# Autodesk Inventor assembly: Pendolo_Inverso
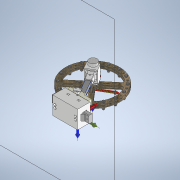
[picture p0: Inventor's stored thumbnail of the model, 180x180]
Saved by Autodesk Inventor 2020.2 (Build 242310000, 310)
## iProperties
Created: 2019-11-10
Part Number: Pendolo_Inverso
Document SubType Name: Assembly
Designer: socci
Author: socci
## Documents named in this file (27)
- C:\Users\socci\Desktop\mv-Project\04_PartDraw\Pendolo_Inverso.iam
- C:\Users\socci\Desktop\mv-Project\04_PartDraw\Componenti\19_Base_Pezzo_Unico.ipt
- C:\Users\socci\Documents\Inventor\Content Center Files\R2020\it-IT\Bearing GB_T 5800-2003\Rolling bearing GB_T 5800-2003 -635.ipt
- C:\Users\socci\Desktop\mv-Project\04_PartDraw\Componenti\1_Asse_cuscinetti.ipt
- C:\Users\socci\Desktop\mv-Project\04_PartDraw\Componenti\2_Connettore_inf_sup.ipt
- C:\Users\socci\Desktop\mv-Project\04_PartDraw\Componenti\3_Connettore_inf_INF.ipt
- C:\Users\socci\Desktop\mv-Project\04_PartDraw\Componenti\11_Connettore_MPU.ipt
- C:\Users\socci\Desktop\mv-Project\04_PartDraw\Componenti\10_MPU_6050.ipt
- C:\Users\socci\Desktop\mv-Project\04_PartDraw\Componenti\20_Base_Sopra.ipt
- C:\Users\socci\Desktop\mv-Project\04_PartDraw\Componenti\4_barra.ipt
- C:\Users\socci\Desktop\mv-Project\04_PartDraw\Componenti\22_Blocco_Escursione_Braccio.ipt
- C:\Users\socci\Desktop\mv-Project\04_PartDraw\Componenti\9_Flangia.ipt
- C:\Users\socci\Desktop\mv-Project\04_PartDraw\Componenti\24_Disco.ipt
- C:\Users\socci\Desktop\mv-Project\04_PartDraw\Componenti\26_Collana_di_Sfere.ipt
- C:\Users\socci\Documents\Inventor\Content Center Files\R2020\it-IT\DIN 1587\DIN 1587 - M6 x 1.ipt
- C:\Users\socci\Documents\Inventor\Content Center Files\R2020\it-IT\DIN 934\DIN 934 - M6 x 1.ipt
- C:\Users\socci\Desktop\mv-Project\04_PartDraw\Componenti\28_Rondella_M6.ipt
- C:\Users\socci\Documents\Inventor\Content Center Files\R2020\it-IT\DIN 933\DIN 933 - M6  x 30.ipt
- C:\Users\socci\Desktop\mv-Project\04_PartDraw\Componenti\30_Connettore_sup.ipt
- C:\Users\socci\Desktop\mv-Project\04_PartDraw\Componenti\29_Motore_6mm.ipt
- C:\Users\socci\Desktop\mv-Project\04_PartDraw\Componenti\0_Sistemariferimento.ipt
- C:\Users\socci\Documents\Inventor\Content Center Files\R2020\it-IT\UNI 5739\UNI 5739 - M5 x 40.ipt
- C:\Users\socci\Documents\Inventor\Content Center Files\R2020\it-IT\IS 2016  A\IS 2016 - A5,5.ipt
- C:\Users\socci\Documents\Inventor\Content Center Files\R2020\it-IT\AS 1112 (4)\AS 1112 - M5(2).ipt
- C:\Users\socci\Documents\Inventor\Content Center Files\R2020\it-IT\AS 1110\AS 1110 - M3 x 25.ipt
- C:\Users\socci\Documents\Inventor\Content Center Files\R2020\it-IT\AS 1237 (2.1)\AS 1237 - 3.ipt
- C:\Users\socci\Documents\Inventor\Content Center Files\R2020\it-IT\AS 1112 (2)\AS 1112 - M3  Tipo 5.ipt
## Components (210 placed, 26 different names)
1. 19_Base_Pezzo_Unico:1 — Inserimento:1, Inserimento:2, Angolo:1, Coincidente:3, Coincidente:4, Coincidente:11, Coincidente:12, Allineato:4, Coincidente:14, Coincidente:15, Allineato:5, Inserimento:323, Inserimento:327, Inserimento:331, Inserimento:335, Coincidente:28, Allineato:6, Allineato:7, Coincidente:29
2. Bearing GB/T 5800-2003 635:1 — Inserimento:1, Inserimento:3, Inserimento:9
3. Bearing GB/T 5800-2003 635:2 — Inserimento:2, Inserimento:4, Inserimento:8
4. 1_Asse_cuscinetti:1 — Inserimento:3, Inserimento:4, Inserimento:5, Inserimento:6, Inserimento:7
5. 2_Connettore_inf_sup:1 — Inserimento:6, Coincidente:1, Angolo:1, Allineato:3, Coincidente:5, Coincidente:6, Coincidente:7, Inserimento:337, Inserimento:338, Inserimento:341, Inserimento:342, Inserimento:345, Inserimento:346, Inserimento:349, Inserimento:350
6. 3_Connettore_inf_INF:1 — Inserimento:5, Coincidente:1, Inserimento:343, Inserimento:347, Inserimento:351
7. 11_Connettore_MPU:1 — Coincidente:2, Allineato:1, Allineato:2, Allineato:3, Inserimento:7
8. 10_MPU_6050:1 — Coincidente:2, Allineato:1, Allineato:2
9. 20_Base_Sopra:1 — Coincidente:3, Inserimento:9, Inserimento:321, Inserimento:322, Inserimento:325, Inserimento:326
10. 20_Base_Sopra:2 — Coincidente:4, Inserimento:8, Inserimento:329, Inserimento:330, Inserimento:333, Inserimento:334
11. 4_barra:1 — Coincidente:5, Coincidente:6, Coincidente:7, Coincidente:19, Coincidente:20, Coincidente:21
12. 22_Blocco_Escursione_Braccio:1 — Coincidente:11, Coincidente:12, Allineato:4
13. 22_Blocco_Escursione_Braccio:2 — Coincidente:14, Coincidente:15, Allineato:5
14. 9_Flangia:1 — Coincidente:24, Inserimento:354, Inserimento:356, Inserimento:358, Inserimento:359
15. 30_Connettore_sup:1 — Coincidente:19, Coincidente:20, Coincidente:21, Inserimento:318, Inserimento:319, Allineato:9, Coincidente:30
16. 29_Motore_6mm:1 — Inserimento:318, Inserimento:319, Inserimento:359
17. 0_Sistemariferimento:1 — Allineato:6, Allineato:7, Coincidente:29
18. 0_Sistemariferimento:2 — Allineato:8, Allineato:9, Coincidente:30, Coincidente:31, Allineato:10, Allineato:11
19. 0_Sistemariferimento:3 — Coincidente:31, Allineato:10, Allineato:11
20. 24_Disco:1 — Inserimento:352, Inserimento:353, Inserimento:355, Inserimento:357, Allineato:8
21. 24_Disco:2 — Inserimento:316, Inserimento:317
22. DIN 1587 M6:1
23. DIN 934 - sostituito da DIN EN 24032/28673/28674 M6:1
24. 28_Rondella_M6:1
25. DIN 933 - sostituito da DIN EN 24017 M6  x 30:1
26. 28_Rondella_M6:2
27. 28_Rondella_M6:3
28. 28_Rondella_M6:4
29. 28_Rondella_M6:5
30. 28_Rondella_M6:6
31. DIN 1587 M6:2
32. DIN 934 - sostituito da DIN EN 24032/28673/28674 M6:2
33. 28_Rondella_M6:7
34. DIN 933 - sostituito da DIN EN 24017 M6  x 30:2
35. 28_Rondella_M6:8
36. 28_Rondella_M6:9
37. 28_Rondella_M6:10
38. 28_Rondella_M6:11
39. 28_Rondella_M6:12
40. DIN 1587 M6:3
41. DIN 934 - sostituito da DIN EN 24032/28673/28674 M6:3
42. 28_Rondella_M6:13
43. DIN 933 - sostituito da DIN EN 24017 M6  x 30:3
44. 28_Rondella_M6:14
45. 28_Rondella_M6:15
46. 28_Rondella_M6:16
47. 28_Rondella_M6:17
48. 28_Rondella_M6:18
49. DIN 1587 M6:4
50. DIN 934 - sostituito da DIN EN 24032/28673/28674 M6:4
51. 28_Rondella_M6:19
52. DIN 933 - sostituito da DIN EN 24017 M6  x 30:4
53. 28_Rondella_M6:20
54. 28_Rondella_M6:21
55. 28_Rondella_M6:22
56. 28_Rondella_M6:23
57. 28_Rondella_M6:24
58. DIN 1587 M6:5
59. DIN 934 - sostituito da DIN EN 24032/28673/28674 M6:5
60. 28_Rondella_M6:25
61. DIN 933 - sostituito da DIN EN 24017 M6  x 30:5
62. 28_Rondella_M6:26
63. 28_Rondella_M6:27
64. 28_Rondella_M6:28
65. 28_Rondella_M6:29
66. 28_Rondella_M6:30
67. DIN 1587 M6:6
68. DIN 934 - sostituito da DIN EN 24032/28673/28674 M6:6
69. 28_Rondella_M6:31
70. DIN 933 - sostituito da DIN EN 24017 M6  x 30:6
71. 28_Rondella_M6:32
72. 28_Rondella_M6:33
73. 28_Rondella_M6:34
74. 28_Rondella_M6:35
75. 28_Rondella_M6:36
76. DIN 1587 M6:7
77. DIN 934 - sostituito da DIN EN 24032/28673/28674 M6:7
78. 28_Rondella_M6:37
79. DIN 933 - sostituito da DIN EN 24017 M6  x 30:7
80. 28_Rondella_M6:38
81. 28_Rondella_M6:39
82. 28_Rondella_M6:40
83. 28_Rondella_M6:41
84. 28_Rondella_M6:42
85. DIN 1587 M6:8
86. DIN 934 - sostituito da DIN EN 24032/28673/28674 M6:8
87. 28_Rondella_M6:43
88. DIN 933 - sostituito da DIN EN 24017 M6  x 30:8
89. 28_Rondella_M6:44
90. 28_Rondella_M6:45
91. 28_Rondella_M6:46
92. 28_Rondella_M6:47
93. 28_Rondella_M6:48
94. DIN 1587 M6:9
95. DIN 934 - sostituito da DIN EN 24032/28673/28674 M6:9
96. 28_Rondella_M6:49
97. DIN 933 - sostituito da DIN EN 24017 M6  x 30:9
98. 28_Rondella_M6:50
99. 28_Rondella_M6:51
100. 28_Rondella_M6:52
101. 28_Rondella_M6:53
102. 28_Rondella_M6:54
103. DIN 1587 M6:10
104. DIN 934 - sostituito da DIN EN 24032/28673/28674 M6:10
105. 28_Rondella_M6:55
106. DIN 933 - sostituito da DIN EN 24017 M6  x 30:10
107. 28_Rondella_M6:56
108. 28_Rondella_M6:57
109. 28_Rondella_M6:58
110. 28_Rondella_M6:59
111. 28_Rondella_M6:60
112. DIN 1587 M6:11
113. DIN 934 - sostituito da DIN EN 24032/28673/28674 M6:11
114. 28_Rondella_M6:61
115. DIN 933 - sostituito da DIN EN 24017 M6  x 30:11
116. 28_Rondella_M6:62
117. 28_Rondella_M6:63
118. 28_Rondella_M6:64
119. 28_Rondella_M6:65
120. 28_Rondella_M6:66
121. DIN 1587 M6:12
122. DIN 934 - sostituito da DIN EN 24032/28673/28674 M6:12
123. 28_Rondella_M6:67
124. DIN 933 - sostituito da DIN EN 24017 M6  x 30:12
125. 28_Rondella_M6:68
126. 28_Rondella_M6:69
127. 28_Rondella_M6:70
128. 28_Rondella_M6:71
129. 28_Rondella_M6:72
130. DIN 1587 M6:13
131. DIN 934 - sostituito da DIN EN 24032/28673/28674 M6:13
132. 28_Rondella_M6:73
133. DIN 933 - sostituito da DIN EN 24017 M6  x 30:13
134. 28_Rondella_M6:74
135. 28_Rondella_M6:75
136. 28_Rondella_M6:76
137. 28_Rondella_M6:77
138. 28_Rondella_M6:78
139. DIN 1587 M6:14
140. DIN 934 - sostituito da DIN EN 24032/28673/28674 M6:14
141. 28_Rondella_M6:79
142. DIN 933 - sostituito da DIN EN 24017 M6  x 30:14
143. 28_Rondella_M6:80
144. 28_Rondella_M6:81
145. 28_Rondella_M6:82
146. 28_Rondella_M6:83
147. 28_Rondella_M6:84
148. DIN 1587 M6:15
149. DIN 934 - sostituito da DIN EN 24032/28673/28674 M6:15
150. 28_Rondella_M6:85
151. DIN 933 - sostituito da DIN EN 24017 M6  x 30:15
152. 28_Rondella_M6:86
153. 28_Rondella_M6:87
154. 28_Rondella_M6:88
155. 28_Rondella_M6:89
156. 28_Rondella_M6:90
157. DIN 1587 M6:16
158. DIN 934 - sostituito da DIN EN 24032/28673/28674 M6:16
159. 28_Rondella_M6:91
160. DIN 933 - sostituito da DIN EN 24017 M6  x 30:16
161. 28_Rondella_M6:92
162. 28_Rondella_M6:93
163. 28_Rondella_M6:94
164. 28_Rondella_M6:95
165. 28_Rondella_M6:96
166. 26_Collana_di_Sfere:1 — Inserimento:316, Inserimento:317
167. AS 1237 (2.1) 3:1 — Coincidente:23
168. AS 1110 - Metrico M3 x 25:1 — Coincidente:23, Inserimento:352
169. AS 1112 (2) - Metrico M3  Tipo 5:1 — Coincidente:24
170. AS 1110 - Metrico M3 x 25:2
171. AS 1237 (2.1) 3:2 — Inserimento:353
172. AS 1112 (2) - Metrico M3  Tipo 5:2 — Inserimento:354
173. AS 1110 - Metrico M3 x 25:3
174. AS 1237 (2.1) 3:3 — Inserimento:355
175. AS 1112 (2) - Metrico M3  Tipo 5:3 — Inserimento:356
176. AS 1110 - Metrico M3 x 25:4
177. AS 1237 (2.1) 3:4 — Inserimento:357
178. AS 1112 (2) - Metrico M3  Tipo 5:4 — Inserimento:358
179. UNI 5739 M5 x 40:4 — Inserimento:320
180. IS 2016 A A5,5:7 — Inserimento:322
181. IS 2016 A A5,5:8 — Inserimento:320, Inserimento:321
182. AS 1112 (4) - Metrico M5:1 — Inserimento:323
183. UNI 5739 M5 x 40:5
184. IS 2016 A A5,5:9 — Inserimento:326
185. IS 2016 A A5,5:10 — Inserimento:325
186. AS 1112 (4) - Metrico M5:2 — Inserimento:327
187. UNI 5739 M5 x 40:6
188. IS 2016 A A5,5:11 — Inserimento:330
189. IS 2016 A A5,5:12 — Inserimento:329
190. AS 1112 (4) - Metrico M5:3 — Inserimento:331
191. UNI 5739 M5 x 40:7
192. IS 2016 A A5,5:13 — Inserimento:334
193. IS 2016 A A5,5:14 — Inserimento:333
194. AS 1112 (4) - Metrico M5:4 — Inserimento:335
195. UNI 5739 M5 x 40:8 — Inserimento:339
196. IS 2016 A A5,5:15 — Inserimento:338
197. IS 2016 A A5,5:16 — Inserimento:337
198. AS 1112 (4) - Metrico M5:5 — Inserimento:339
199. UNI 5739 M5 x 40:9
200. IS 2016 A A5,5:17 — Inserimento:342
201. IS 2016 A A5,5:18 — Inserimento:341
202. AS 1112 (4) - Metrico M5:6 — Inserimento:343
203. UNI 5739 M5 x 40:10
204. IS 2016 A A5,5:19 — Inserimento:346
205. IS 2016 A A5,5:20 — Inserimento:345
206. AS 1112 (4) - Metrico M5:7 — Inserimento:347
207. UNI 5739 M5 x 40:11
208. IS 2016 A A5,5:21 — Inserimento:350
209. IS 2016 A A5,5:22 — Inserimento:349
210. AS 1112 (4) - Metrico M5:8 — Inserimento:351
## Relationships (239: Insert 203, Mate 24, Flush 11, Angle 1)
- Inserimento:1: 19_Base_Pezzo_Unico:1 ↔ Bearing GB/T 5800-2003 635:1
- Inserimento:2: 19_Base_Pezzo_Unico:1 ↔ Bearing GB/T 5800-2003 635:2
- Inserimento:3 (1.5 mm): Bearing GB/T 5800-2003 635:1 ↔ 1_Asse_cuscinetti:1
- Inserimento:4 (2.5 mm): Bearing GB/T 5800-2003 635:2 ↔ 1_Asse_cuscinetti:1
- Inserimento:5: 1_Asse_cuscinetti:1 ↔ 3_Connettore_inf_INF:1
- Inserimento:6: 1_Asse_cuscinetti:1 ↔ 2_Connettore_inf_sup:1
- Coincidente:1 [Mate] (1 mm): 2_Connettore_inf_sup:1 ↔ 3_Connettore_inf_INF:1
- Coincidente:2 [Mate] (10 mm): 11_Connettore_MPU:1 ↔ 10_MPU_6050:1
- Allineato:1 [Flush] (2 mm): 11_Connettore_MPU:1 ↔ 10_MPU_6050:1
- Allineato:2 [Flush] (3 mm): 11_Connettore_MPU:1 ↔ 10_MPU_6050:1
- Angolo:1 [Angle] (-30 deg): 19_Base_Pezzo_Unico:1 ↔ 2_Connettore_inf_sup:1
- Allineato:3 [Flush] (-9.5 mm): 2_Connettore_inf_sup:1 ↔ 11_Connettore_MPU:1
- Inserimento:7: 1_Asse_cuscinetti:1 ↔ 11_Connettore_MPU:1
- Coincidente:3 [Mate] (1 mm): 19_Base_Pezzo_Unico:1 ↔ 20_Base_Sopra:1
- Coincidente:4 [Mate] (1 mm): 19_Base_Pezzo_Unico:1 ↔ 20_Base_Sopra:2
- Inserimento:8: Bearing GB/T 5800-2003 635:2 ↔ 20_Base_Sopra:2
- Inserimento:9: Bearing GB/T 5800-2003 635:1 ↔ 20_Base_Sopra:1
- Coincidente:5 [Mate] (0.5 mm): 2_Connettore_inf_sup:1 ↔ 4_barra:1
- Coincidente:6 [Mate] (0.5 mm): 2_Connettore_inf_sup:1 ↔ 4_barra:1
- Coincidente:7 [Mate]: 2_Connettore_inf_sup:1 ↔ 4_barra:1
- Coincidente:11 [Mate]: 19_Base_Pezzo_Unico:1 ↔ 22_Blocco_Escursione_Braccio:1
- Coincidente:12 [Mate] (0.2 mm): 19_Base_Pezzo_Unico:1 ↔ 22_Blocco_Escursione_Braccio:1
- Allineato:4 [Flush]: 19_Base_Pezzo_Unico:1 ↔ 22_Blocco_Escursione_Braccio:1
- Coincidente:14 [Mate] (0.2 mm): 19_Base_Pezzo_Unico:1 ↔ 22_Blocco_Escursione_Braccio:2
- Coincidente:15 [Mate]: 19_Base_Pezzo_Unico:1 ↔ 22_Blocco_Escursione_Braccio:2
- Allineato:5 [Flush]: 19_Base_Pezzo_Unico:1 ↔ 22_Blocco_Escursione_Braccio:2
- [Insert] (7.829 mm): 24_Disco:1 ↔ 24_Disco:2
- [Insert] (7.829 mm): 24_Disco:1 ↔ 24_Disco:2
- [Insert] (7.829 mm): 24_Disco:1 ↔ 24_Disco:2
- [Insert] (7.829 mm): 24_Disco:1 ↔ 24_Disco:2
- [Insert]: 28_Rondella_M6:1 ↔ DIN 933 - sostituito da DIN EN 24017 M6  x 30:1
- [Insert] (4 mm): 28_Rondella_M6:1 ↔ 28_Rondella_M6:2
- [Insert]: DIN 934 - sostituito da DIN EN 24032/28673/28674 M6:1 ↔ 28_Rondella_M6:2
- [Insert]: DIN 934 - sostituito da DIN EN 24032/28673/28674 M6:1 ↔ 28_Rondella_M6:3
- [Insert] (4 mm): 28_Rondella_M6:3 ↔ 28_Rondella_M6:5
- [Insert]: 28_Rondella_M6:5 ↔ 28_Rondella_M6:6
- [Insert]: 28_Rondella_M6:4 ↔ 28_Rondella_M6:6
- [Insert]: DIN 1587 M6:1 ↔ 28_Rondella_M6:4
- [Insert]: 28_Rondella_M6:7 ↔ DIN 933 - sostituito da DIN EN 24017 M6  x 30:2
- [Insert] (4 mm): 28_Rondella_M6:7 ↔ 28_Rondella_M6:8
- [Insert]: DIN 934 - sostituito da DIN EN 24032/28673/28674 M6:2 ↔ 28_Rondella_M6:8
- [Insert]: DIN 934 - sostituito da DIN EN 24032/28673/28674 M6:2 ↔ 28_Rondella_M6:9
- [Insert] (4 mm): 28_Rondella_M6:9 ↔ 28_Rondella_M6:11
- [Insert]: 28_Rondella_M6:11 ↔ 28_Rondella_M6:12
- [Insert]: 28_Rondella_M6:10 ↔ 28_Rondella_M6:12
- [Insert]: DIN 1587 M6:2 ↔ 28_Rondella_M6:10
- [Insert]: 24_Disco:2 ↔ 28_Rondella_M6:7
- [Insert]: 28_Rondella_M6:13 ↔ DIN 933 - sostituito da DIN EN 24017 M6  x 30:3
- [Insert] (4 mm): 28_Rondella_M6:13 ↔ 28_Rondella_M6:14
- [Insert]: DIN 934 - sostituito da DIN EN 24032/28673/28674 M6:3 ↔ 28_Rondella_M6:14
- [Insert]: DIN 934 - sostituito da DIN EN 24032/28673/28674 M6:3 ↔ 28_Rondella_M6:15
- [Insert] (4 mm): 28_Rondella_M6:15 ↔ 28_Rondella_M6:17
- [Insert]: 28_Rondella_M6:17 ↔ 28_Rondella_M6:18
- [Insert]: 28_Rondella_M6:16 ↔ 28_Rondella_M6:18
- [Insert]: DIN 1587 M6:3 ↔ 28_Rondella_M6:16
- [Insert]: 28_Rondella_M6:19 ↔ DIN 933 - sostituito da DIN EN 24017 M6  x 30:4
- [Insert] (4 mm): 28_Rondella_M6:19 ↔ 28_Rondella_M6:20
- [Insert]: DIN 934 - sostituito da DIN EN 24032/28673/28674 M6:4 ↔ 28_Rondella_M6:20
- [Insert]: DIN 934 - sostituito da DIN EN 24032/28673/28674 M6:4 ↔ 28_Rondella_M6:21
- [Insert] (4 mm): 28_Rondella_M6:21 ↔ 28_Rondella_M6:23
- [Insert]: 28_Rondella_M6:23 ↔ 28_Rondella_M6:24
- [Insert]: 28_Rondella_M6:22 ↔ 28_Rondella_M6:24
- [Insert]: DIN 1587 M6:4 ↔ 28_Rondella_M6:22
- [Insert]: 28_Rondella_M6:25 ↔ DIN 933 - sostituito da DIN EN 24017 M6  x 30:5
- [Insert] (4 mm): 28_Rondella_M6:25 ↔ 28_Rondella_M6:26
- [Insert]: DIN 934 - sostituito da DIN EN 24032/28673/28674 M6:5 ↔ 28_Rondella_M6:26
- [Insert]: DIN 934 - sostituito da DIN EN 24032/28673/28674 M6:5 ↔ 28_Rondella_M6:27
- [Insert] (4 mm): 28_Rondella_M6:27 ↔ 28_Rondella_M6:29
- [Insert]: 28_Rondella_M6:29 ↔ 28_Rondella_M6:30
- [Insert]: 28_Rondella_M6:28 ↔ 28_Rondella_M6:30
- [Insert]: DIN 1587 M6:5 ↔ 28_Rondella_M6:28
- [Insert]: 28_Rondella_M6:31 ↔ DIN 933 - sostituito da DIN EN 24017 M6  x 30:6
- [Insert] (4 mm): 28_Rondella_M6:31 ↔ 28_Rondella_M6:32
- [Insert]: DIN 934 - sostituito da DIN EN 24032/28673/28674 M6:6 ↔ 28_Rondella_M6:32
- [Insert]: DIN 934 - sostituito da DIN EN 24032/28673/28674 M6:6 ↔ 28_Rondella_M6:33
- [Insert] (4 mm): 28_Rondella_M6:33 ↔ 28_Rondella_M6:35
- [Insert]: 28_Rondella_M6:35 ↔ 28_Rondella_M6:36
- [Insert]: 28_Rondella_M6:34 ↔ 28_Rondella_M6:36
- [Insert]: DIN 1587 M6:6 ↔ 28_Rondella_M6:34
- [Insert]: 28_Rondella_M6:37 ↔ DIN 933 - sostituito da DIN EN 24017 M6  x 30:7
- [Insert] (4 mm): 28_Rondella_M6:37 ↔ 28_Rondella_M6:38
- [Insert]: DIN 934 - sostituito da DIN EN 24032/28673/28674 M6:7 ↔ 28_Rondella_M6:38
- [Insert]: DIN 934 - sostituito da DIN EN 24032/28673/28674 M6:7 ↔ 28_Rondella_M6:39
- [Insert] (4 mm): 28_Rondella_M6:39 ↔ 28_Rondella_M6:41
- [Insert]: 28_Rondella_M6:41 ↔ 28_Rondella_M6:42
- [Insert]: 28_Rondella_M6:40 ↔ 28_Rondella_M6:42
- [Insert]: DIN 1587 M6:7 ↔ 28_Rondella_M6:40
- [Insert]: 28_Rondella_M6:43 ↔ DIN 933 - sostituito da DIN EN 24017 M6  x 30:8
- [Insert] (4 mm): 28_Rondella_M6:43 ↔ 28_Rondella_M6:44
- [Insert]: DIN 934 - sostituito da DIN EN 24032/28673/28674 M6:8 ↔ 28_Rondella_M6:44
- [Insert]: DIN 934 - sostituito da DIN EN 24032/28673/28674 M6:8 ↔ 28_Rondella_M6:45
- [Insert] (4 mm): 28_Rondella_M6:45 ↔ 28_Rondella_M6:47
- [Insert]: 28_Rondella_M6:47 ↔ 28_Rondella_M6:48
- [Insert]: 28_Rondella_M6:46 ↔ 28_Rondella_M6:48
- [Insert]: DIN 1587 M6:8 ↔ 28_Rondella_M6:46
- [Insert]: 28_Rondella_M6:49 ↔ DIN 933 - sostituito da DIN EN 24017 M6  x 30:9
- [Insert] (4 mm): 28_Rondella_M6:49 ↔ 28_Rondella_M6:50
- [Insert]: DIN 934 - sostituito da DIN EN 24032/28673/28674 M6:9 ↔ 28_Rondella_M6:50
- [Insert]: DIN 934 - sostituito da DIN EN 24032/28673/28674 M6:9 ↔ 28_Rondella_M6:51
- [Insert] (4 mm): 28_Rondella_M6:51 ↔ 28_Rondella_M6:53
- [Insert]: 28_Rondella_M6:53 ↔ 28_Rondella_M6:54
- [Insert]: 28_Rondella_M6:52 ↔ 28_Rondella_M6:54
- [Insert]: DIN 1587 M6:9 ↔ 28_Rondella_M6:52
- [Insert]: 28_Rondella_M6:55 ↔ DIN 933 - sostituito da DIN EN 24017 M6  x 30:10
- [Insert] (4 mm): 28_Rondella_M6:55 ↔ 28_Rondella_M6:56
- [Insert]: DIN 934 - sostituito da DIN EN 24032/28673/28674 M6:10 ↔ 28_Rondella_M6:56
- [Insert]: DIN 934 - sostituito da DIN EN 24032/28673/28674 M6:10 ↔ 28_Rondella_M6:57
- [Insert] (4 mm): 28_Rondella_M6:57 ↔ 28_Rondella_M6:59
- [Insert]: 28_Rondella_M6:59 ↔ 28_Rondella_M6:60
- [Insert]: 28_Rondella_M6:58 ↔ 28_Rondella_M6:60
- [Insert]: DIN 1587 M6:10 ↔ 28_Rondella_M6:58
- [Insert]: 28_Rondella_M6:61 ↔ DIN 933 - sostituito da DIN EN 24017 M6  x 30:11
- [Insert] (4 mm): 28_Rondella_M6:61 ↔ 28_Rondella_M6:62
- [Insert]: DIN 934 - sostituito da DIN EN 24032/28673/28674 M6:11 ↔ 28_Rondella_M6:62
- [Insert]: DIN 934 - sostituito da DIN EN 24032/28673/28674 M6:11 ↔ 28_Rondella_M6:63
- [Insert] (4 mm): 28_Rondella_M6:63 ↔ 28_Rondella_M6:65
- [Insert]: 28_Rondella_M6:65 ↔ 28_Rondella_M6:66
- [Insert]: 28_Rondella_M6:64 ↔ 28_Rondella_M6:66
- [Insert]: DIN 1587 M6:11 ↔ 28_Rondella_M6:64
- [Insert]: 28_Rondella_M6:67 ↔ DIN 933 - sostituito da DIN EN 24017 M6  x 30:12
- [Insert] (4 mm): 28_Rondella_M6:67 ↔ 28_Rondella_M6:68
- [Insert]: DIN 934 - sostituito da DIN EN 24032/28673/28674 M6:12 ↔ 28_Rondella_M6:68
- [Insert]: DIN 934 - sostituito da DIN EN 24032/28673/28674 M6:12 ↔ 28_Rondella_M6:69
- [Insert] (4 mm): 28_Rondella_M6:69 ↔ 28_Rondella_M6:71
- [Insert]: 28_Rondella_M6:71 ↔ 28_Rondella_M6:72
- [Insert]: 28_Rondella_M6:70 ↔ 28_Rondella_M6:72
- [Insert]: DIN 1587 M6:12 ↔ 28_Rondella_M6:70
- [Insert]: 28_Rondella_M6:73 ↔ DIN 933 - sostituito da DIN EN 24017 M6  x 30:13
- [Insert] (4 mm): 28_Rondella_M6:73 ↔ 28_Rondella_M6:74
- [Insert]: DIN 934 - sostituito da DIN EN 24032/28673/28674 M6:13 ↔ 28_Rondella_M6:74
- [Insert]: DIN 934 - sostituito da DIN EN 24032/28673/28674 M6:13 ↔ 28_Rondella_M6:75
- [Insert] (4 mm): 28_Rondella_M6:75 ↔ 28_Rondella_M6:77
- [Insert]: 28_Rondella_M6:77 ↔ 28_Rondella_M6:78
- [Insert]: 28_Rondella_M6:76 ↔ 28_Rondella_M6:78
- [Insert]: DIN 1587 M6:13 ↔ 28_Rondella_M6:76
- [Insert]: 28_Rondella_M6:79 ↔ DIN 933 - sostituito da DIN EN 24017 M6  x 30:14
- [Insert] (4 mm): 28_Rondella_M6:79 ↔ 28_Rondella_M6:80
- [Insert]: DIN 934 - sostituito da DIN EN 24032/28673/28674 M6:14 ↔ 28_Rondella_M6:80
- [Insert]: DIN 934 - sostituito da DIN EN 24032/28673/28674 M6:14 ↔ 28_Rondella_M6:81
- [Insert] (4 mm): 28_Rondella_M6:81 ↔ 28_Rondella_M6:83
- [Insert]: 28_Rondella_M6:83 ↔ 28_Rondella_M6:84
- [Insert]: 28_Rondella_M6:82 ↔ 28_Rondella_M6:84
- [Insert]: DIN 1587 M6:14 ↔ 28_Rondella_M6:82
- [Insert]: 28_Rondella_M6:85 ↔ DIN 933 - sostituito da DIN EN 24017 M6  x 30:15
- [Insert] (4 mm): 28_Rondella_M6:85 ↔ 28_Rondella_M6:86
- [Insert]: DIN 934 - sostituito da DIN EN 24032/28673/28674 M6:15 ↔ 28_Rondella_M6:86
- [Insert]: DIN 934 - sostituito da DIN EN 24032/28673/28674 M6:15 ↔ 28_Rondella_M6:87
- [Insert] (4 mm): 28_Rondella_M6:87 ↔ 28_Rondella_M6:89
- [Insert]: 28_Rondella_M6:89 ↔ 28_Rondella_M6:90
- [Insert]: 28_Rondella_M6:88 ↔ 28_Rondella_M6:90
- [Insert]: DIN 1587 M6:15 ↔ 28_Rondella_M6:88
- [Insert]: 28_Rondella_M6:91 ↔ DIN 933 - sostituito da DIN EN 24017 M6  x 30:16
- [Insert] (4 mm): 28_Rondella_M6:91 ↔ 28_Rondella_M6:92
- [Insert]: DIN 934 - sostituito da DIN EN 24032/28673/28674 M6:16 ↔ 28_Rondella_M6:92
- [Insert]: DIN 934 - sostituito da DIN EN 24032/28673/28674 M6:16 ↔ 28_Rondella_M6:93
- [Insert] (4 mm): 28_Rondella_M6:93 ↔ 28_Rondella_M6:95
- [Insert]: 28_Rondella_M6:95 ↔ 28_Rondella_M6:96
- [Insert]: 28_Rondella_M6:94 ↔ 28_Rondella_M6:96
- [Insert]: DIN 1587 M6:16 ↔ 28_Rondella_M6:94
- [Insert]: 24_Disco:2 ↔ 28_Rondella_M6:1
- [Insert]: 24_Disco:2 ↔ 28_Rondella_M6:91
- [Insert]: 24_Disco:2 ↔ 28_Rondella_M6:19
- [Insert]: 24_Disco:2 ↔ 28_Rondella_M6:43
- [Insert]: 24_Disco:2 ↔ 28_Rondella_M6:49
- [Insert]: 24_Disco:2 ↔ 28_Rondella_M6:55
- [Insert]: 24_Disco:2 ↔ 28_Rondella_M6:67
- [Insert]: 24_Disco:2 ↔ 28_Rondella_M6:79
- [Insert]: 24_Disco:2 ↔ 28_Rondella_M6:85
- [Insert]: 24_Disco:2 ↔ 28_Rondella_M6:73
- [Insert]: 24_Disco:2 ↔ 28_Rondella_M6:37
- [Insert]: 24_Disco:2 ↔ 28_Rondella_M6:61
- [Insert]: 24_Disco:2 ↔ 28_Rondella_M6:25
- [Insert]: 24_Disco:2 ↔ 28_Rondella_M6:13
- [Insert]: 24_Disco:2 ↔ 28_Rondella_M6:31
- [Mate]: 9_Flangia:1 ↔ 24_Disco:2
- [Insert]: 9_Flangia:1 ↔ 24_Disco:2
- [Insert]: 9_Flangia:1 ↔ 24_Disco:2
- Inserimento:316: 24_Disco:2 ↔ 26_Collana_di_Sfere:1
- Inserimento:317: 24_Disco:2 ↔ 26_Collana_di_Sfere:1
- Coincidente:19 [Mate]: 4_barra:1 ↔ 30_Connettore_sup:1
- Coincidente:20 [Mate]: 4_barra:1 ↔ 30_Connettore_sup:1
- Coincidente:21 [Mate]: 4_barra:1 ↔ 30_Connettore_sup:1
- Inserimento:318: 30_Connettore_sup:1 ↔ 29_Motore_6mm:1
- Inserimento:319: 30_Connettore_sup:1 ↔ 29_Motore_6mm:1
- Inserimento:320: UNI 5739 M5 x 40:4 ↔ IS 2016 A A5,5:8
- Inserimento:321: 20_Base_Sopra:1 ↔ IS 2016 A A5,5:8
- Inserimento:322: 20_Base_Sopra:1 ↔ IS 2016 A A5,5:7
- Inserimento:323: 19_Base_Pezzo_Unico:1 ↔ AS 1112 (4) - Metrico M5:1
- [Insert]: UNI 5739 M5 x 40:5 ↔ IS 2016 A A5,5:10
- Inserimento:325: 20_Base_Sopra:1 ↔ IS 2016 A A5,5:10
- Inserimento:326: 20_Base_Sopra:1 ↔ IS 2016 A A5,5:9
- Inserimento:327: 19_Base_Pezzo_Unico:1 ↔ AS 1112 (4) - Metrico M5:2
- [Insert]: UNI 5739 M5 x 40:6 ↔ IS 2016 A A5,5:12
- Inserimento:329: 20_Base_Sopra:2 ↔ IS 2016 A A5,5:12
- Inserimento:330: 20_Base_Sopra:2 ↔ IS 2016 A A5,5:11
- Inserimento:331: 19_Base_Pezzo_Unico:1 ↔ AS 1112 (4) - Metrico M5:3
- [Insert]: UNI 5739 M5 x 40:7 ↔ IS 2016 A A5,5:14
- Inserimento:333: 20_Base_Sopra:2 ↔ IS 2016 A A5,5:14
- Inserimento:334: 20_Base_Sopra:2 ↔ IS 2016 A A5,5:13
- Inserimento:335: 19_Base_Pezzo_Unico:1 ↔ AS 1112 (4) - Metrico M5:4
- [Insert]: UNI 5739 M5 x 40:8 ↔ IS 2016 A A5,5:16
- Inserimento:337: 2_Connettore_inf_sup:1 ↔ IS 2016 A A5,5:16
- Inserimento:338: 2_Connettore_inf_sup:1 ↔ IS 2016 A A5,5:15
- Inserimento:339: UNI 5739 M5 x 40:8 ↔ AS 1112 (4) - Metrico M5:5
- [Insert]: UNI 5739 M5 x 40:9 ↔ IS 2016 A A5,5:18
- Inserimento:341: 2_Connettore_inf_sup:1 ↔ IS 2016 A A5,5:18
- Inserimento:342: 2_Connettore_inf_sup:1 ↔ IS 2016 A A5,5:17
- Inserimento:343: 3_Connettore_inf_INF:1 ↔ AS 1112 (4) - Metrico M5:6
- [Insert]: UNI 5739 M5 x 40:10 ↔ IS 2016 A A5,5:20
- Inserimento:345: 2_Connettore_inf_sup:1 ↔ IS 2016 A A5,5:20
- Inserimento:346: 2_Connettore_inf_sup:1 ↔ IS 2016 A A5,5:19
- Inserimento:347: 3_Connettore_inf_INF:1 ↔ AS 1112 (4) - Metrico M5:7
- [Insert]: UNI 5739 M5 x 40:11 ↔ IS 2016 A A5,5:22
- Inserimento:349: 2_Connettore_inf_sup:1 ↔ IS 2016 A A5,5:22
- Inserimento:350: 2_Connettore_inf_sup:1 ↔ IS 2016 A A5,5:21
- Inserimento:351: 3_Connettore_inf_INF:1 ↔ AS 1112 (4) - Metrico M5:8
- Coincidente:23 [Mate]: AS 1237 (2.1) 3:1 ↔ AS 1110 - Metrico M3 x 25:1
- Inserimento:352: 24_Disco:1 ↔ AS 1110 - Metrico M3 x 25:1
- Coincidente:24 [Mate]: 9_Flangia:1 ↔ AS 1112 (2) - Metrico M3  Tipo 5:1
- [Mate]: AS 1110 - Metrico M3 x 25:2 ↔ AS 1237 (2.1) 3:2
- Inserimento:353: 24_Disco:1 ↔ AS 1237 (2.1) 3:2
- Inserimento:354: 9_Flangia:1 ↔ AS 1112 (2) - Metrico M3  Tipo 5:2
- [Mate]: AS 1110 - Metrico M3 x 25:3 ↔ AS 1237 (2.1) 3:3
- Inserimento:355: 24_Disco:1 ↔ AS 1237 (2.1) 3:3
- Inserimento:356: 9_Flangia:1 ↔ AS 1112 (2) - Metrico M3  Tipo 5:3
- [Mate]: AS 1110 - Metrico M3 x 25:4 ↔ AS 1237 (2.1) 3:4
- Inserimento:357: 24_Disco:1 ↔ AS 1237 (2.1) 3:4
- Inserimento:358: 9_Flangia:1 ↔ AS 1112 (2) - Metrico M3  Tipo 5:4
- Coincidente:28 [Mate]: 19_Base_Pezzo_Unico:1
- Inserimento:359: 9_Flangia:1 ↔ 29_Motore_6mm:1
- Allineato:6 [Flush] (36 mm): 19_Base_Pezzo_Unico:1 ↔ 0_Sistemariferimento:1
- Allineato:7 [Flush] (96 mm): 19_Base_Pezzo_Unico:1 ↔ 0_Sistemariferimento:1
- Coincidente:29 [Mate] (96 mm): 19_Base_Pezzo_Unico:1 ↔ 0_Sistemariferimento:1
- Allineato:8 [Flush] (106 mm): 0_Sistemariferimento:2 ↔ 24_Disco:1
- Allineato:9 [Flush] (71.45 mm): 30_Connettore_sup:1 ↔ 0_Sistemariferimento:2
- Coincidente:30 [Mate] (71.8 mm): 30_Connettore_sup:1 ↔ 0_Sistemariferimento:2
- Coincidente:31 [Mate]: 0_Sistemariferimento:2 ↔ 0_Sistemariferimento:3
- Allineato:10 [Flush]: 0_Sistemariferimento:2 ↔ 0_Sistemariferimento:3
- Allineato:11 [Flush] (-192 mm): 0_Sistemariferimento:2 ↔ 0_Sistemariferimento:3
## Named parameters: d362_d2 = 7.829 mm, d363_d3 = 7.829 mm, d103_d6 = 0 mm, d104_d7 = 4 mm, d105_d8 = 0 mm, d106_d9 = 0 mm, d107_d10 = 4 mm, d108_d11 = 0 mm, d109_d12 = 0 mm, d110_d13 = 0 mm, d111_d6 = 0 mm, d112_d7 = 4 mm, d113_d8 = 0 mm, d114_d9 = 0 mm, d115_d10 = 4 mm, d116_d11 = 0 mm, d117_d12 = 0 mm, d118_d13 = 0 mm, d119_d6 = 0 mm, d120_d7 = 4 mm, d121_d8 = 0 mm, d122_d9 = 0 mm, d123_d10 = 4 mm, d124_d11 = 0 mm, d125_d12 = 0 mm, d126_d13 = 0 mm, d127_d6 = 0 mm, d128_d7 = 4 mm, d129_d8 = 0 mm, d130_d9 = 0 mm, d131_d10 = 4 mm, d132_d11 = 0 mm, d133_d12 = 0 mm, d134_d13 = 0 mm, d65_d8 = 0 mm, d66_d9 = 0 mm, d67_d10 = 4 mm, d68_d11 = 0 mm, d69_d12 = 0 mm, d70_d13 = 0 mm, d71_d6 = 0 mm, d72_d7 = 4 mm, d73_d8 = 0 mm, d74_d9 = 0 mm, d75_d10 = 4 mm, d76_d11 = 0 mm, d77_d12 = 0 mm, d78_d13 = 0 mm, d79_d6 = 0 mm, d80_d7 = 4 mm, d81_d8 = 0 mm, d82_d9 = 0 mm, d83_d10 = 4 mm, d84_d11 = 0 mm, d85_d12 = 0 mm, d86_d13 = 0 mm, d87_d6 = 0 mm, d88_d7 = 4 mm, d89_d8 = 0 mm, d90_d9 = 0 mm, d91_d10 = 4 mm, d92_d11 = 0 mm, d93_d12 = 0 mm, d94_d13 = 0 mm, d95_d6 = 0 mm, d96_d7 = 4 mm, d97_d8 = 0 mm, d98_d9 = 0 mm, d99_d10 = 4 mm, d100_d11 = 0 mm, d101_d12 = 0 mm, d102_d13 = 0 mm, d31_d6 = 0 mm, d32_d7 = 4 mm, d33_d8 = 0 mm, d34_d9 = 0 mm, d35_d10 = 4 mm, d36_d11 = 0 mm, d37_d12 = 0 mm, d38_d13 = 0 mm, d39_d6 = 0 mm, d40_d7 = 4 mm, d41_d8 = 0 mm, d42_d9 = 0 mm, d43_d10 = 4 mm, d44_d11 = 0 mm, d45_d12 = 0 mm, d46_d13 = 0 mm, d47_d6 = 0 mm, d48_d7 = 4 mm, d49_d8 = 0 mm, d50_d9 = 0 mm, d51_d10 = 4 mm, d52_d11 = 0 mm, d53_d12 = 0 mm, d54_d13 = 0 mm, d55_d6 = 0 mm, d56_d7 = 4 mm, d57_d8 = 0 mm, d58_d9 = 0 mm, d59_d10 = 4 mm, d60_d11 = 0 mm, d61_d12 = 0 mm, d62_d13 = 0 mm, d63_d6 = 0 mm, d64_d7 = 4 mm, d485_d6 = 0 mm, d486_d7 = 4 mm, d487_d8 = 0 mm, d489_d10 = 4 mm, d490_d11 = 0 mm, d491_d12 = 0 mm, d492_d13 = 0 mm, d14_d6 = 0 mm, d15_d7 = 4 mm, d16_d8 = 0 mm, d17_d9 = 0 mm, d18_d10 = 4 mm, d19_d11 = 0 mm, d20_d12 = 0 mm, d21_d13 = 0 mm, d501_d22 = 0 mm, d23_d6 = 0 mm, d24_d7 = 4 mm, d25_d8 = 0 mm, d26_d9 = 0 mm, d27_d10 = 4 mm, d28_d11 = 0 mm, d29_d12 = 0 mm, d30_d13 = 0 mm, d522_d518 = 0 mm, d526_d518 = 0 mm, d530_d518 = 0 mm, d535_d530_d518 = 0 mm, d539_d530_d518 = 0 mm, d543_d530_d518 = 0 mm, d547_d530_d518 = 0 mm, d554_d551 = 0 mm, d557_d551 = 0 mm, d560_d551 = 0 mm
